# Autodesk Inventor assembly: ASM1001-16bit-CPU.git
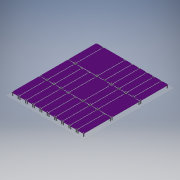
[picture p0: Inventor's stored thumbnail of the model, 180x180]
Saved by Autodesk Inventor 2019 (Build 230136000, 136)
## iProperties
Created: 2019-07-02
Part Number: ASM1001-16bit-CPU.git
Document SubType Name: Assembly
Designer: james
Author: james
## Documents named in this file (5)
- F:\JimsDesign\P1001-16bit-CPU\P1001-001 - 16bit CPU\ASM1001-16bit-CPU.git.iam
- F:\JimsDesign\P1001-16bit-CPU\P1001-001 - 16bit CPU\PRT1001-213 Base.ipt
- F:\JimsDesign\P1001-16bit-CPU\P1001-001 - 16bit CPU\ASM1001-210 1U Board.iam
- F:\JimsDesign\P1001-16bit-CPU\P1001-001 - 16bit CPU\ASM1001-211 2U Board.iam
- F:\JimsDesign\P1001-16bit-CPU\P1001-001 - 16bit CPU\ASM1001-212 3U Board.iam
## Components (27 placed, 4 different names)
1. PRT1001-213 Base:1 — Mate:1, Mate:2, Mate:3, Mate:4, Mate:5, Mate:6, Mate:7, Mate:8, Mate:9, Mate:10, Mate:11, Mate:12, Mate:13, Mate:14, Mate:15, Mate:16, Mate:17, Mate:18, Mate:19, Mate:20, Mate:21, Mate:22, Mate:23, Mate:24, Mate:25, Mate:26, Mate:27, Mate:28, Mate:29, Mate:30, Mate:31, Mate:32, Mate:33, Mate:34, Mate:35, Mate:36, Mate:37, Mate:38, Mate:39, Mate:40, Mate:41, Mate:42, Mate:43, Mate:44, Mate:45, Mate:46, Mate:47, Mate:48, Mate:49, Mate:50, Mate:51, Mate:52, Mate:53, Mate:54, Mate:55, Mate:56, Mate:57
2. ASM1001-210 1U Board:1 [sub-assembly] — Mate:7, Mate:8, Mate:9, Flush:6
3. ASM1001-210 1U Board:2 [sub-assembly] — Flush:1, Mate:18, Mate:19, Flush:2, Flush:3
4. ASM1001-210 1U Board:3 [sub-assembly] — Mate:15, Mate:16, Mate:17, Flush:1
5. ASM1001-210 1U Board:4 [sub-assembly] — Mate:12, Mate:13, Mate:14, Flush:4
6. ASM1001-210 1U Board:5 [sub-assembly] — Mate:10, Mate:11, Flush:5
7. ASM1001-210 1U Board:6 [sub-assembly] — Mate:1, Mate:2, Mate:3
8. ASM1001-210 1U Board:7 [sub-assembly] — Mate:4, Mate:5, Mate:6, Flush:7, Flush:8
9. ASM1001-210 1U Board:8 [sub-assembly] — Flush:8, Mate:26, Mate:30, Flush:9
10. ASM1001-210 1U Board:9 [sub-assembly] — Flush:7, Mate:24, Mate:25
11. ASM1001-210 1U Board:10 [sub-assembly] — Flush:6, Mate:29, Mate:33
12. ASM1001-210 1U Board:11 [sub-assembly] — Flush:5, Mate:22, Mate:23
13. ASM1001-210 1U Board:12 [sub-assembly] — Flush:4, Mate:27, Mate:31, Flush:10
14. ASM1001-210 1U Board:13 [sub-assembly] — Flush:3, Mate:20, Mate:21
15. ASM1001-210 1U Board:14 [sub-assembly] — Flush:2, Mate:28, Mate:32
16. ASM1001-210 1U Board:15 [sub-assembly] — Flush:9, Mate:34, Mate:35
17. ASM1001-211 2U Board:1 [sub-assembly] — Flush:10, Mate:36, Mate:37, Flush:11, Flush:12, Flush:13, Flush:14
18. ASM1001-212 3U Board:1 [sub-assembly] — Flush:11, Mate:38, Mate:39, Flush:15, Flush:16, Flush:17, Flush:18
19. ASM1001-210 1U Board:16 [sub-assembly] — Flush:17, Mate:40, Mate:43
20. ASM1001-210 1U Board:17 [sub-assembly] — Flush:16, Mate:41, Mate:44
21. ASM1001-210 1U Board:18 [sub-assembly] — Flush:15, Mate:47, Mate:51
22. ASM1001-210 1U Board:19 [sub-assembly] — Flush:18, Mate:46, Mate:50
23. ASM1001-210 1U Board:20 [sub-assembly] — Flush:14, Mate:48, Mate:52
24. ASM1001-210 1U Board:21 [sub-assembly] — Flush:13, Mate:49, Mate:53, Flush:19, Flush:20
25. ASM1001-211 2U Board:3 [sub-assembly] — Flush:12, Mate:42, Mate:45
26. ASM1001-210 1U Board:22 [sub-assembly] — Flush:20, Mate:54, Mate:56
27. ASM1001-210 1U Board:23 [sub-assembly] — Flush:19, Mate:55, Mate:57
## Relationships (77: Mate 57, Flush 20)
- Mate:1: PRT1001-213 Base:1 ↔ ASM1001-210 1U Board:6
- Mate:2: PRT1001-213 Base:1 ↔ ASM1001-210 1U Board:6
- Mate:3: PRT1001-213 Base:1 ↔ ASM1001-210 1U Board:6
- Mate:4: PRT1001-213 Base:1 ↔ ASM1001-210 1U Board:7
- Mate:5: PRT1001-213 Base:1 ↔ ASM1001-210 1U Board:7
- Mate:6: PRT1001-213 Base:1 ↔ ASM1001-210 1U Board:7
- Mate:7: PRT1001-213 Base:1 ↔ ASM1001-210 1U Board:1
- Mate:8: PRT1001-213 Base:1 ↔ ASM1001-210 1U Board:1
- Mate:9: PRT1001-213 Base:1 ↔ ASM1001-210 1U Board:1
- Mate:10: PRT1001-213 Base:1 ↔ ASM1001-210 1U Board:5
- Mate:11: PRT1001-213 Base:1 ↔ ASM1001-210 1U Board:5
- Mate:12: PRT1001-213 Base:1 ↔ ASM1001-210 1U Board:4
- Mate:13: PRT1001-213 Base:1 ↔ ASM1001-210 1U Board:4
- Mate:14: PRT1001-213 Base:1 ↔ ASM1001-210 1U Board:4
- Mate:15: PRT1001-213 Base:1 ↔ ASM1001-210 1U Board:3
- Mate:16: PRT1001-213 Base:1 ↔ ASM1001-210 1U Board:3
- Mate:17: PRT1001-213 Base:1 ↔ ASM1001-210 1U Board:3
- Flush:1: ASM1001-210 1U Board:2 ↔ ASM1001-210 1U Board:3
- Mate:18: PRT1001-213 Base:1 ↔ ASM1001-210 1U Board:2
- Mate:19: PRT1001-213 Base:1 ↔ ASM1001-210 1U Board:2
- Flush:2: ASM1001-210 1U Board:2 ↔ ASM1001-210 1U Board:14
- Flush:3: ASM1001-210 1U Board:2 ↔ ASM1001-210 1U Board:13
- Flush:4: ASM1001-210 1U Board:4 ↔ ASM1001-210 1U Board:12
- Flush:5: ASM1001-210 1U Board:5 ↔ ASM1001-210 1U Board:11
- Flush:6: ASM1001-210 1U Board:1 ↔ ASM1001-210 1U Board:10
- Flush:7: ASM1001-210 1U Board:7 ↔ ASM1001-210 1U Board:9
- Flush:8: ASM1001-210 1U Board:7 ↔ ASM1001-210 1U Board:8
- Mate:20: PRT1001-213 Base:1 ↔ ASM1001-210 1U Board:13
- Mate:21: PRT1001-213 Base:1 ↔ ASM1001-210 1U Board:13
- Mate:22: PRT1001-213 Base:1 ↔ ASM1001-210 1U Board:11
- Mate:23: PRT1001-213 Base:1 ↔ ASM1001-210 1U Board:11
- Mate:24: PRT1001-213 Base:1 ↔ ASM1001-210 1U Board:9
- Mate:25: PRT1001-213 Base:1 ↔ ASM1001-210 1U Board:9
- Mate:26: PRT1001-213 Base:1 ↔ ASM1001-210 1U Board:8
- Mate:27: PRT1001-213 Base:1 ↔ ASM1001-210 1U Board:12
- Mate:28: PRT1001-213 Base:1 ↔ ASM1001-210 1U Board:14
- Mate:29: PRT1001-213 Base:1 ↔ ASM1001-210 1U Board:10
- Mate:30: PRT1001-213 Base:1 ↔ ASM1001-210 1U Board:8
- Mate:31: PRT1001-213 Base:1 ↔ ASM1001-210 1U Board:12
- Mate:32: PRT1001-213 Base:1 ↔ ASM1001-210 1U Board:14
- Mate:33: PRT1001-213 Base:1 ↔ ASM1001-210 1U Board:10
- Flush:9: ASM1001-210 1U Board:8 ↔ ASM1001-210 1U Board:15
- Flush:10: ASM1001-210 1U Board:12 ↔ ASM1001-211 2U Board:1
- Mate:34: PRT1001-213 Base:1 ↔ ASM1001-210 1U Board:15
- Mate:35: PRT1001-213 Base:1 ↔ ASM1001-210 1U Board:15
- Mate:36: PRT1001-213 Base:1 ↔ ASM1001-211 2U Board:1
- Mate:37: PRT1001-213 Base:1 ↔ ASM1001-211 2U Board:1
- Flush:11: ASM1001-211 2U Board:1 ↔ ASM1001-212 3U Board:1
- Mate:38: PRT1001-213 Base:1 ↔ ASM1001-212 3U Board:1
- Mate:39: PRT1001-213 Base:1 ↔ ASM1001-212 3U Board:1
- Flush:12: ASM1001-211 2U Board:1 ↔ ASM1001-211 2U Board:3
- Flush:13: ASM1001-211 2U Board:1 ↔ ASM1001-210 1U Board:21
- Flush:14: ASM1001-211 2U Board:1 ↔ ASM1001-210 1U Board:20
- Flush:15: ASM1001-212 3U Board:1 ↔ ASM1001-210 1U Board:18
- Flush:16: ASM1001-212 3U Board:1 ↔ ASM1001-210 1U Board:17
- Flush:17: ASM1001-212 3U Board:1 ↔ ASM1001-210 1U Board:16
- Mate:40: PRT1001-213 Base:1 ↔ ASM1001-210 1U Board:16
- Mate:41: PRT1001-213 Base:1 ↔ ASM1001-210 1U Board:17
- Mate:42: PRT1001-213 Base:1 ↔ ASM1001-211 2U Board:3
- Mate:43: PRT1001-213 Base:1 ↔ ASM1001-210 1U Board:16
- Mate:44: PRT1001-213 Base:1 ↔ ASM1001-210 1U Board:17
- Mate:45: PRT1001-213 Base:1 ↔ ASM1001-211 2U Board:3
- Flush:18: ASM1001-212 3U Board:1 ↔ ASM1001-210 1U Board:19
- Mate:46: PRT1001-213 Base:1 ↔ ASM1001-210 1U Board:19
- Mate:47: PRT1001-213 Base:1 ↔ ASM1001-210 1U Board:18
- Mate:48: PRT1001-213 Base:1 ↔ ASM1001-210 1U Board:20
- Mate:49: PRT1001-213 Base:1 ↔ ASM1001-210 1U Board:21
- Mate:50: PRT1001-213 Base:1 ↔ ASM1001-210 1U Board:19
- Mate:51: PRT1001-213 Base:1 ↔ ASM1001-210 1U Board:18
- Mate:52: PRT1001-213 Base:1 ↔ ASM1001-210 1U Board:20
- Mate:53: PRT1001-213 Base:1 ↔ ASM1001-210 1U Board:21
- Flush:19: ASM1001-210 1U Board:21 ↔ ASM1001-210 1U Board:23
- Flush:20: ASM1001-210 1U Board:21 ↔ ASM1001-210 1U Board:22
- Mate:54: PRT1001-213 Base:1 ↔ ASM1001-210 1U Board:22
- Mate:55: PRT1001-213 Base:1 ↔ ASM1001-210 1U Board:23
- Mate:56: PRT1001-213 Base:1 ↔ ASM1001-210 1U Board:22
- Mate:57: PRT1001-213 Base:1 ↔ ASM1001-210 1U Board:23
